# Autodesk Inventor assembly: Assemblynew
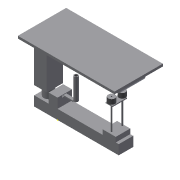
[picture p0: Inventor's stored thumbnail of the model, 180x180]
Saved by Autodesk Inventor 2019 (Build 230136000, 136)
## iProperties
Created: 2019-11-25
Part Number: Assemblynew
Document SubType Name: Assembly
Designer: Mahesh
Author: Mahesh
## Documents named in this file (5)
- F:\Assemblynew.iam
- F:\Part6.ipt
- F:\Part9.ipt
- F:\new part ee.ipt
- F:\new part ee.2.ipt
## Components (4 placed, 4 different names)
1. Part6:1 — Insert:1
2. Part9:1 — Insert:1, Insert:2
3. new part ee:1 — Insert:2
4. new part ee.2:1
## Relationships (2: Insert 2)
- Insert:1: Part6:1 ↔ Part9:1
- Insert:2: Part9:1 ↔ new part ee:1
